# Autodesk Inventor assembly: testerscrew
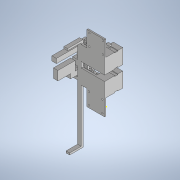
[picture p0: Inventor's stored thumbnail of the model, 180x180]
Saved by Autodesk Inventor 2020.2 (Build 242310000, 310)
## iProperties
Created: 2020-02-28
Part Number: testerscrew
Document SubType Name: Assembly
Designer: ColinP
Author: ColinP
## Documents named in this file (9)
- C:\Users\ColinP\Documents\Inventor\steppermotoriqc\SteppermotorLaser\testerscrew.iam
- C:\Users\ColinP\Documents\Inventor\steppermotoriqc\SteppermotorLaser\shell 1.0 screw top.ipt
- C:\Users\ColinP\Documents\Inventor\steppermotoriqc\95462A029_GRADE 5 STEEL HEX NUT.ipt
- C:\Users\ColinP\Documents\Inventor\steppermotoriqc\28BYJ-48 – 5V Stepper Motor\28BYJ-48 – 5V Stepper Motor.ipt
- C:\Users\ColinP\Documents\Inventor\steppermotoriqc\SteppermotorLaser\lever.ipt
- C:\Users\ColinP\Documents\Inventor\steppermotoriqc\SteppermotorLaser\lever staggered.ipt
- C:\Users\ColinP\Documents\Inventor\steppermotoriqc\SteppermotorLaser\shell 2.0 screw.ipt
- C:\Users\ColinP\Documents\Inventor\steppermotoriqc\SteppermotorLaser\4.ipt
- C:\Users\ColinP\Documents\Inventor\Content Center Files\R2020\en-US\ANSI B18.3(05)\ANSI B18.3 - 1_4-20 UNC - 0.75(31).ipt
## Components (15 placed, 8 different names)
1. shell 1.0 screw top:1 — Mate:1, Mate:2, Mate:3, Mate:4, Mate:23
2. shell 2.0 screw:1 — Mate:1, Mate:2, Mate:3, Mate:5, Mate:9, Mate:10, Mate:11, Mate:14, Mate:16, Mate:17, Mate:18, Mate:19, Mate:20, Mate:21, Mate:22, Mate:39, Mate:40
3. 95462A029_GRADE 5 STEEL HEX NUT:1 — Mate:4, Mate:5, Mate:23
4. 28BYJ-48 – 5V Stepper Motor:1 — Mate:9, Mate:10, Mate:11, Mate:27, Mate:28
5. lever:2 — Mate:14
6. lever staggered:1 — Mate:16
7. shell 1.0 screw top:2 — Mate:17, Mate:18, Mate:19, Mate:38
8. 28BYJ-48 – 5V Stepper Motor:2 — Mate:20, Mate:21, Mate:22, Mate:32, Mate:33
9. 4:1 — Mate:24, Mate:25, Mate:26, Mate:28, Mate:34, Mate:35
10. 4:2 — Mate:24, Mate:25, Mate:26, Mate:27
11. 4:3 — Mate:29, Mate:30, Mate:31, Mate:32, Mate:33, Mate:36
12. 4:4 — Mate:29, Mate:30, Mate:31, Mate:37
13. Hexagon Socket Head Cap Screw - Inch 1/4 - 20 UNC - 3/4:1 — Mate:34, Mate:35
14. Hexagon Socket Head Cap Screw - Inch 1/4 - 20 UNC - 3/4:2 — Mate:36, Mate:37
15. 95462A029_GRADE 5 STEEL HEX NUT:2 — Mate:38, Mate:39, Mate:40
## Relationships (34: Mate 34)
- Mate:1: shell 1.0 screw top:1 ↔ shell 2.0 screw:1
- Mate:2: shell 1.0 screw top:1 ↔ shell 2.0 screw:1
- Mate:3: shell 1.0 screw top:1 ↔ shell 2.0 screw:1
- Mate:4: shell 1.0 screw top:1 ↔ 95462A029_GRADE 5 STEEL HEX NUT:1
- Mate:5: shell 2.0 screw:1 ↔ 95462A029_GRADE 5 STEEL HEX NUT:1
- Mate:9: shell 2.0 screw:1 ↔ 28BYJ-48 – 5V Stepper Motor:1
- Mate:10: shell 2.0 screw:1 ↔ 28BYJ-48 – 5V Stepper Motor:1
- Mate:11: shell 2.0 screw:1 ↔ 28BYJ-48 – 5V Stepper Motor:1
- Mate:14: shell 2.0 screw:1 ↔ lever:2
- Mate:16: shell 2.0 screw:1 ↔ lever staggered:1
- Mate:17: shell 2.0 screw:1 ↔ shell 1.0 screw top:2
- Mate:18: shell 2.0 screw:1 ↔ shell 1.0 screw top:2
- Mate:19: shell 2.0 screw:1 ↔ shell 1.0 screw top:2
- Mate:20: shell 2.0 screw:1 ↔ 28BYJ-48 – 5V Stepper Motor:2
- Mate:21: shell 2.0 screw:1 ↔ 28BYJ-48 – 5V Stepper Motor:2
- Mate:22: shell 2.0 screw:1 ↔ 28BYJ-48 – 5V Stepper Motor:2
- Mate:23: shell 1.0 screw top:1 ↔ 95462A029_GRADE 5 STEEL HEX NUT:1
- Mate:24: 4:1 ↔ 4:2
- Mate:25: 4:1 ↔ 4:2
- Mate:26: 4:1 ↔ 4:2
- Mate:27: 28BYJ-48 – 5V Stepper Motor:1 ↔ 4:2
- Mate:28: 28BYJ-48 – 5V Stepper Motor:1 ↔ 4:1
- Mate:29: 4:3 ↔ 4:4
- Mate:30: 4:3 ↔ 4:4
- Mate:31: 4:3 ↔ 4:4
- Mate:32: 28BYJ-48 – 5V Stepper Motor:2 ↔ 4:3
- Mate:33: 28BYJ-48 – 5V Stepper Motor:2 ↔ 4:3
- Mate:34: 4:1 ↔ Hexagon Socket Head Cap Screw - Inch 1/4 - 20 UNC - 3/4:1
- Mate:35: 4:1 ↔ Hexagon Socket Head Cap Screw - Inch 1/4 - 20 UNC - 3/4:1
- Mate:36: 4:3 ↔ Hexagon Socket Head Cap Screw - Inch 1/4 - 20 UNC - 3/4:2
- Mate:37: 4:4 ↔ Hexagon Socket Head Cap Screw - Inch 1/4 - 20 UNC - 3/4:2
- Mate:38: shell 1.0 screw top:2 ↔ 95462A029_GRADE 5 STEEL HEX NUT:2
- Mate:39: shell 2.0 screw:1 ↔ 95462A029_GRADE 5 STEEL HEX NUT:2
- Mate:40: shell 2.0 screw:1 ↔ 95462A029_GRADE 5 STEEL HEX NUT:2
